# Autodesk Inventor assembly: Mount_v0.1.0_Assembly
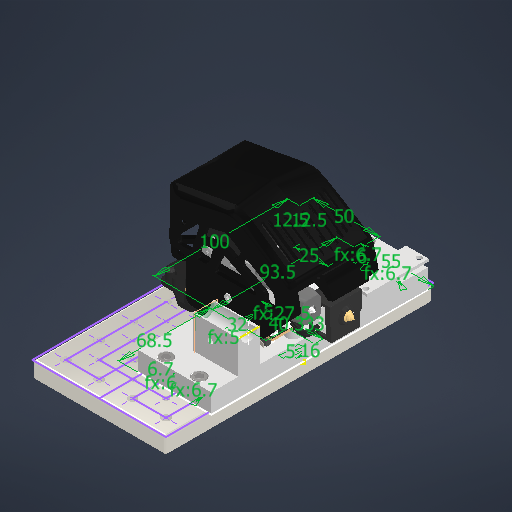
[picture p0: Inventor's stored thumbnail of the model, 512x512]
Saved by Autodesk Inventor 2027 (Build 310192060, 192F)
## iProperties
Created: 2026-07-09
Part Number: Mount_v0.1.0_Assembly
Document SubType Name: Assembly
Designer: jacob
Author: jacob
## Documents named in this file (10)
- C:\Users\jacob\Documents\Autodesk\Inventor 2027\mount_proj_v3\Mount_v0.1.1_Assembly.iam
- Mount_v0.1.0_Assembly.iam
- C:\Users\jacob\Documents\Autodesk\Inventor 2027\mount_proj_v3\Base_Plate.ipt
- C:\Users\jacob\Documents\Autodesk\Inventor 2027\mount_proj_v3\Mount_v0.1.1.ipt
- C:\Users\jacob\OneDrive\Documents\Inventor\Content Center Files\R2027\en-US\ANSI B18.3.1M(6)\ANSI B18.3.1M - M6x1 x 12(1).ipt
- C:\Users\jacob\Documents\Autodesk\Inventor 2027\mount_proj_v3\M5_Bolt_Derived.ipt
- C:\Users\jacob\Documents\Autodesk\Inventor 2027\mount_proj_v3\M5_Nut_Derived.ipt
- C:\Users\jacob\Documents\Autodesk\Inventor 2027\mount_proj_v3\Ender_3_V3_SE_Derived.ipt
- C:\Users\jacob\Documents\Autodesk\Inventor 2027\mount_proj_v3\ILD1x20-500.ipt
- C:\Users\jacob\Documents\Autodesk\Inventor 2027\mount_proj_v3\thermoMETER UC.ipt
## Components (15 placed, 8 different names)
1. Base_Plate:1 — Mate:1, Mate:2, Angle:1
2. Mount_v0.1.0 — Mate:1, Mate:2, Mate:3, Mate:4, Mate:5, Mate:6, Rotational:4, Rotational:5, Rotational:6, Rotational:7, Rotational:8, Rotational:9, Rotational:10
3. Ender_3_V3_SE_Derived:1 — Mate:6, Angle:1, Rotational:1, Rotational:2, Rotational:3
4. ILD1x20-500:1 — Mate:3, Mate:4
5. thermoMETER UC:1 — Mate:5
6. M5_Nut_Derived:1 — Rotational:6
7. M5_Nut_Derived:2 — Rotational:4
8. M5_Nut_Derived:3 — Rotational:5
9. M5_Bolt_Derived:2 — Rotational:3
10. M5_Bolt_Derived:3 — Rotational:1
11. M5_Bolt_Derived:1 — Rotational:2
12. Forged Socket Head Cap Screw - Metric M6x1 x 12:1 — Rotational:8
13. Forged Socket Head Cap Screw - Metric M6x1 x 12:2 — Rotational:9
14. Forged Socket Head Cap Screw - Metric M6x1 x 12:3 — Rotational:10
15. Forged Socket Head Cap Screw - Metric M6x1 x 12:4 — Rotational:7
## Relationships (17: RevoluteJoint 10, Mate 6, Angle 1)
- Mate:1: Base_Plate:1 ↔ Mount_v0.1.0
- Mate:2: Base_Plate:1 ↔ Mount_v0.1.0
- Mate:3: Mount_v0.1.0 ↔ ILD1x20-500:1
- Mate:4: Mount_v0.1.0 ↔ ILD1x20-500:1
- Mate:5: Mount_v0.1.0 ↔ thermoMETER UC:1
- Mate:6: Mount_v0.1.0 ↔ Ender_3_V3_SE_Derived:1
- Angle:1 (0 deg): Base_Plate:1 ↔ Ender_3_V3_SE_Derived:1
- Rotational:1 [RevoluteJoint]: Ender_3_V3_SE_Derived:1 ↔ M5_Bolt_Derived:3
- Rotational:2 [RevoluteJoint]: Ender_3_V3_SE_Derived:1 ↔ M5_Bolt_Derived:1
- Rotational:3 [RevoluteJoint]: Ender_3_V3_SE_Derived:1 ↔ M5_Bolt_Derived:2
- Rotational:4 [RevoluteJoint]: Mount_v0.1.0 ↔ M5_Nut_Derived:2
- Rotational:5 [RevoluteJoint]: Mount_v0.1.0 ↔ M5_Nut_Derived:3
- Rotational:6 [RevoluteJoint]: Mount_v0.1.0 ↔ M5_Nut_Derived:1
- Rotational:7 [RevoluteJoint]: Mount_v0.1.0 ↔ Forged Socket Head Cap Screw - Metric M6x1 x 12:4
- Rotational:8 [RevoluteJoint]: Mount_v0.1.0 ↔ Forged Socket Head Cap Screw - Metric M6x1 x 12:1
- Rotational:9 [RevoluteJoint]: Mount_v0.1.0 ↔ Forged Socket Head Cap Screw - Metric M6x1 x 12:2
- Rotational:10 [RevoluteJoint]: Mount_v0.1.0 ↔ Forged Socket Head Cap Screw - Metric M6x1 x 12:3
